# Autodesk Inventor assembly: Stainless arrangement
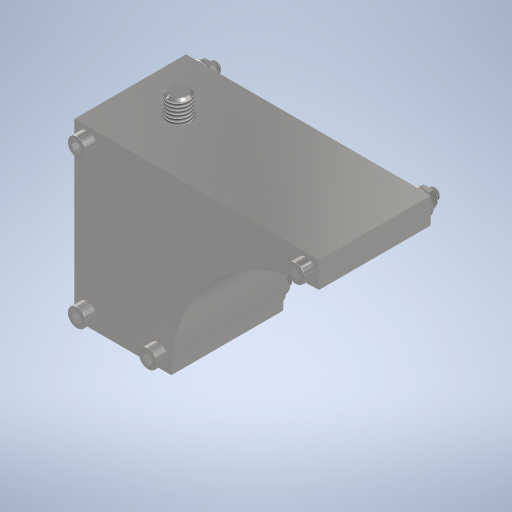
[picture p0: Inventor's stored thumbnail of the model, 512x512]
Saved by Autodesk Inventor 2023 (Build 270158000, 158)
## iProperties
Created: 2023-04-21
Part Number: Stainless arrangement
Document SubType Name: Assembly
Designer: Victoria
Mass: 2269.35 g
Surface Area: 2110.36 cm^2
Volume: 284.047 cm^3
Density: 7.98934 g/cm^3
Author: Victoria
## Documents named in this file (11)
- C:\Users\Valentine\Desktop\Engine supports\Stainless arrangement.iam
- C:\Users\Valentine\Desktop\Engine supports\Stainless sheet support.ipt
- C:\Users\Valentine\Documents\Inventor\Content Center Files\R2023\en-US\CNS 3932\CNS 3932 - M 5 x 0.8 x 60.ipt
- C:\Users\Valentine\Documents\Inventor\Content Center Files\R2023\en-US\ISO 4161\ISO 4161 - M5(1).ipt
- C:\Users\Valentine\Documents\Inventor\Content Center Files\R2023\en-US\ISO 4762(2)\ISO 4762 - M10 x 90ISO.ipt
- C:\Users\Valentine\Desktop\Engine supports\Stainless arrangement\AIP\FEA\eb8423h8g.fins
- C:\Users\Valentine\Desktop\Engine supports\Stainless arrangement\AIP\FEA\eb8423h8g.fsat
- C:\Users\Valentine\Desktop\Engine supports\Stainless arrangement\AIP\FEA\eb8423h8g.ftes
- C:\Users\Valentine\Desktop\Engine supports\Stainless arrangement\AIP\FEA\eb8423h8g.fwiz
- C:\Users\Valentine\Desktop\Engine supports\Stainless arrangement\AIP\FEA\eb8423hb4.fmsh
- C:\Users\Valentine\Desktop\Engine supports\Stainless arrangement\AIP\FEA\eb8423hc0.fres
## Components (26 placed, 4 different names)
1. Stainless sheet support:1 — Mate:12, Mate:14, Mate:58, Mate:82, Mate:88, Mate:92
2. Stainless sheet support:2 — Mate:10, Mate:12, Mate:58, Mate:59, Mate:82
3. Stainless sheet support:3 — Mate:7, Mate:10, Mate:59, Mate:81, Mate:91
4. Stainless sheet support:4 — Mate:16, Mate:18, Mate:37, Mate:65, Mate:83, Mate:93
5. Stainless sheet support:5 — Mate:18, Mate:20, Mate:65, Mate:68, Mate:84, Mate:93
6. Stainless sheet support:6 — Mate:14, Mate:16, Mate:37, Mate:83, Mate:92
7. Stainless sheet support:7 — Mate:32, Mate:34, Mate:36, Mate:87, Mate:98, Mate:99
8. Stainless sheet support:8 — Mate:34, Mate:36, Insert:1, Insert:2, Insert:3, Insert:4, Mate:88, Mate:99
9. Stainless sheet support:9 — Mate:28, Mate:30, Mate:86, Mate:96, Mate:97
10. Stainless sheet support:10 — Mate:30, Mate:32, Mate:87, Mate:97, Mate:98
11. Stainless sheet support:11 — Mate:20, Mate:22, Mate:67, Mate:68, Mate:84
12. Stainless sheet support:12 — Mate:26, Mate:28, Mate:86, Mate:95, Mate:96
13. Stainless sheet support:13 — Mate:1, Mate:4, Mate:80, Mate:89, Mate:90
14. Stainless sheet support:14 — Mate:1, Mate:72, Mate:73, Mate:74, Mate:75, Mate:76, Mate:77, Mate:78, Mate:79, Mate:80, Mate:89
15. Stainless sheet support:15 — Mate:4, Mate:7, Mate:81, Mate:90, Mate:91
16. Stainless sheet support:16 — Mate:22, Mate:24, Mate:67, Mate:85, Mate:94, Insert:5
17. Stainless sheet support:17 — Mate:24, Mate:26, Mate:85, Mate:94, Mate:95
18. CNS 3932 M 5 x 60:1 — Mate:72, Mate:73
19. CNS 3932 M 5 x 60:2 — Mate:74, Mate:75
20. CNS 3932 M 5 x 60:3 — Mate:76, Mate:77
21. CNS 3932 M 5 x 60:4 — Mate:78, Mate:79
22. ISO 4161 M5:1 — Insert:1
23. ISO 4161 M5:2 — Insert:2
24. ISO 4161 M5:3 — Insert:3
25. ISO 4161 M5:4 — Insert:4
26. ISO 4762 M10 x 90:1 — Insert:5
## Relationships (56: Mate 51, Insert 5)
- Mate:1: Stainless sheet support:13 ↔ Stainless sheet support:14
- Mate:4: Stainless sheet support:13 ↔ Stainless sheet support:15
- Mate:7: Stainless sheet support:3 ↔ Stainless sheet support:15
- Mate:10: Stainless sheet support:2 ↔ Stainless sheet support:3
- Mate:12: Stainless sheet support:1 ↔ Stainless sheet support:2
- Mate:14: Stainless sheet support:1 ↔ Stainless sheet support:6
- Mate:16: Stainless sheet support:4 ↔ Stainless sheet support:6
- Mate:18: Stainless sheet support:4 ↔ Stainless sheet support:5
- Mate:20: Stainless sheet support:5 ↔ Stainless sheet support:11
- Mate:22: Stainless sheet support:11 ↔ Stainless sheet support:16
- Mate:24: Stainless sheet support:16 ↔ Stainless sheet support:17
- Mate:26: Stainless sheet support:12 ↔ Stainless sheet support:17
- Mate:28: Stainless sheet support:9 ↔ Stainless sheet support:12
- Mate:30: Stainless sheet support:9 ↔ Stainless sheet support:10
- Mate:32: Stainless sheet support:7 ↔ Stainless sheet support:10
- Mate:34: Stainless sheet support:7 ↔ Stainless sheet support:8
- Mate:36: Stainless sheet support:7 ↔ Stainless sheet support:8
- Mate:37: Stainless sheet support:4 ↔ Stainless sheet support:6
- Mate:58: Stainless sheet support:1 ↔ Stainless sheet support:2
- Mate:59: Stainless sheet support:2 ↔ Stainless sheet support:3
- Mate:65: Stainless sheet support:4 ↔ Stainless sheet support:5
- Mate:67: Stainless sheet support:11 ↔ Stainless sheet support:16
- Mate:68: Stainless sheet support:5 ↔ Stainless sheet support:11
- Mate:72: Stainless sheet support:14 ↔ CNS 3932 M 5 x 60:1
- Mate:73: Stainless sheet support:14 ↔ CNS 3932 M 5 x 60:1
- Mate:74: Stainless sheet support:14 ↔ CNS 3932 M 5 x 60:2
- Mate:75: Stainless sheet support:14 ↔ CNS 3932 M 5 x 60:2
- Mate:76: Stainless sheet support:14 ↔ CNS 3932 M 5 x 60:3
- Mate:77: Stainless sheet support:14 ↔ CNS 3932 M 5 x 60:3
- Mate:78: Stainless sheet support:14 ↔ CNS 3932 M 5 x 60:4
- Mate:79: Stainless sheet support:14 ↔ CNS 3932 M 5 x 60:4
- Insert:1: Stainless sheet support:8 ↔ ISO 4161 M5:1
- Insert:2: Stainless sheet support:8 ↔ ISO 4161 M5:2
- Insert:3: Stainless sheet support:8 ↔ ISO 4161 M5:3
- Insert:4: Stainless sheet support:8 ↔ ISO 4161 M5:4
- Mate:80: Stainless sheet support:13 ↔ Stainless sheet support:14
- Mate:81: Stainless sheet support:3 ↔ Stainless sheet support:15
- Mate:82: Stainless sheet support:1 ↔ Stainless sheet support:2
- Mate:83: Stainless sheet support:4 ↔ Stainless sheet support:6
- Mate:84: Stainless sheet support:5 ↔ Stainless sheet support:11
- Mate:85: Stainless sheet support:16 ↔ Stainless sheet support:17
- Mate:86: Stainless sheet support:9 ↔ Stainless sheet support:12
- Mate:87: Stainless sheet support:7 ↔ Stainless sheet support:10
- Mate:88: Stainless sheet support:1 ↔ Stainless sheet support:8
- Mate:89: Stainless sheet support:13 ↔ Stainless sheet support:14
- Mate:90: Stainless sheet support:13 ↔ Stainless sheet support:15
- Mate:91: Stainless sheet support:3 ↔ Stainless sheet support:15
- Mate:92: Stainless sheet support:1 ↔ Stainless sheet support:6
- Mate:93: Stainless sheet support:4 ↔ Stainless sheet support:5
- Mate:94: Stainless sheet support:16 ↔ Stainless sheet support:17
- Mate:95: Stainless sheet support:12 ↔ Stainless sheet support:17
- Mate:96: Stainless sheet support:9 ↔ Stainless sheet support:12
- Mate:97: Stainless sheet support:9 ↔ Stainless sheet support:10
- Mate:98: Stainless sheet support:7 ↔ Stainless sheet support:10
- Mate:99: Stainless sheet support:7 ↔ Stainless sheet support:8
- Insert:5: Stainless sheet support:16 ↔ ISO 4762 M10 x 90:1
## Named parameters: sa_0 = 200000
note: some values were not read from the file. Shown as the stored number, unit unknown: "sa_0".
